# Autodesk Inventor assembly: FlangeForStorage
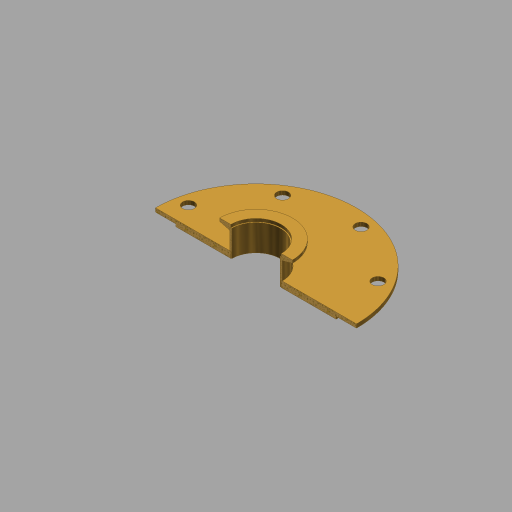
[picture p0: Inventor's stored thumbnail of the model, 512x512]
Saved by Autodesk Inventor 2024 (Build 280153020, 153B)
## iProperties
Created: 2023-11-04
Part Number: FlangeForStorage
Document SubType Name: Assembly
Designer: schanen
Mass: 1790.28 g
Surface Area: 951.935 cm^2
Volume: 213.07 cm^3
Density: 8.40231 g/cm^3
Author: schanen
## Documents named in this file (4)
- C:\Users\schanen\Documents\Inventor\LargeTransportDewarInsert2023\FlangeForStorage.iam
- C:\Users\schanen\Documents\Inventor\LargeTransportDewarInsert2023\Flange.ipt
- C:\Users\schanen\Documents\Inventor\LargeTransportDewarInsert2023\oring.ipt
- C:\Users\schanen\Documents\Inventor\LargeTransportDewarInsert2023\neckForStorage.ipt
## Components (2 placed, 2 different names)
1. Flange:1 — Mate:2, Flush:1
2. neckForStorage:1
## Relationships (4: Mate 3, Flush 1)
- [Mate]: Flange:1 ↔ neckForStorage:1
- Mate:2: Flange:1
- Flush:1: Flange:1
- [Mate]: Flange:1 ↔ neckForStorage:1
## Named parameters: oring_dia = 4 mm
